# Autodesk Inventor assembly: onlyrobot
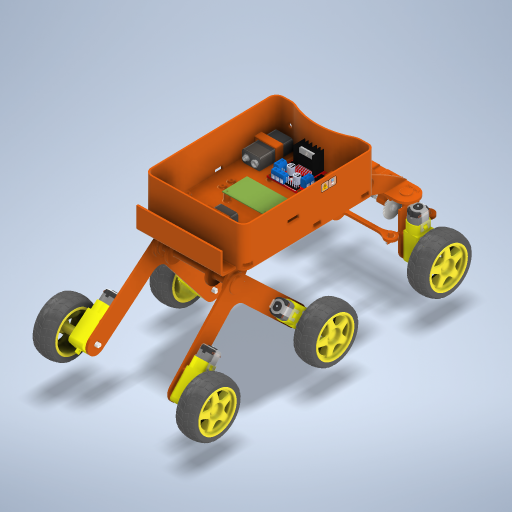
[picture p0: Inventor's stored thumbnail of the model, 512x512]
Saved by Autodesk Inventor 2023.2 (Build 272271000, 271)
## iProperties
Created: 2022-12-08
Part Number: onlyrobot
Document SubType Name: Assembly
Designer: omrfrkmll
Author: omrfrkmll
## Documents named in this file (33)
- C:\Users\omr_f\Desktop\mechanism design project\onlyrobot.iam
- C:\Users\omr_f\Desktop\mechanism design project\robotbase.ipt
- C:\Users\omr_f\Desktop\mechanism design project\sol arka bacak.ipt
- C:\Users\omr_f\Desktop\mechanism design project\6v dc torque motor.iam
- C:\Users\omr_f\Desktop\mechanism design project\Wheel D65x25.ipt
- C:\Users\omr_f\Desktop\mechanism design project\ön sol bacak.ipt
- C:\Users\omr_f\Desktop\mechanism design project\ön sol bacak_MIR.ipt
- C:\Users\omr_f\Desktop\mechanism design project\bişeyleramabendeisimveremedim.ipt
- C:\Users\omr_f\Desktop\mechanism design project\pin.ipt
- C:\Users\omr_f\Desktop\mechanism design project\pintutucu.ipt
- C:\Users\omr_f\Desktop\mechanism design project\pintutucu_MIR.ipt
- C:\Users\omr_f\Desktop\mechanism design project\bilmemç.ipt
- C:\Users\omr_f\Desktop\mechanism design project\Moteur - Moteur.ipt
- C:\Users\omr_f\Desktop\mechanism design project\screw.ipt
- C:\Users\omr_f\Desktop\mechanism design project\dişli.ipt
- C:\Users\omr_f\Desktop\mechanism design project\somun.ipt
- C:\Users\omr_f\Desktop\mechanism design project\benniyebuçüklerinsiminibilmiyorum.ipt
- C:\Users\omr_f\Desktop\mechanism design project\ufakpin.ipt
- C:\Users\omr_f\Desktop\mechanism design project\rockerbogieçükü.ipt
- C:\Users\omr_f\Desktop\mechanism design project\6v dc torque motor_MIR.iam
- C:\Users\omr_f\Desktop\mechanism design project\Wheel D65x25_MIR.ipt
- C:\Users\omr_f\Desktop\mechanism design project\rockerbogieçükü_MIR.ipt
- C:\Users\omr_f\Desktop\mechanism design project\çıkçık.ipt
- C:\Users\omr_f\Desktop\mechanism design project\çıkçıkkarşılıkk.ipt
- C:\Users\omr_f\Desktop\mechanism design project\L298N Driver DC Motor.ipt
- C:\Users\omr_f\Desktop\mechanism design project\devre kartı.ipt
- C:\Users\omr_f\Desktop\mechanism design project\9 Volt Battery.ipt
- C:\Users\omr_f\Desktop\mechanism design project\direksiyon mili tutucu.ipt
- C:\Users\omr_f\Desktop\mechanism design project\şaftuzun.ipt
- C:\Users\omr_f\Desktop\mechanism design project\ön differansiyel.ipt
- C:\Users\omr_f\Desktop\mechanism design project\sol arka bacak_MIR.ipt
- C:\Users\omr_f\Desktop\mechanism design project\onlyrobot\Design Accelerator\Spur Gears2.iam
- C:\Users\omr_f\Desktop\mechanism design project\destek bağlantısı.ipt
## Components (50 placed, 32 different names)
1. robotbase:1 — Mate:87, Mate:88, Mate:89, Mate:90, Mate:91, Mate:92, Mate:94, Mate:95, Mate:96, Mate:97, Mate:99, Mate:100, Mate:101, Mate:102, Mate:103, Mate:113, Mate:114, Mate:115, Mate:120, Mate:121, Mate:122
2. 6v dc torque motor:1 [sub-assembly]
3. Wheel D65x25:1
4. ön sol bacak:1 — Mate:126
5. ön sol bacak_MIR:1 — Mate:133
6. 6v dc torque motor:2 [sub-assembly]
7. Wheel D65x25:2
8. bişeyleramabendeisimveremedim:1 — Flush:1
9. pin:1
10. pintutucu:1 — Mate:106, Mate:110, Mate:111, Mate:112
11. pintutucu_MIR:1 — Mate:105, Mate:109
12. pin:2
13. bilmemç:1 — Mate:104, Mate:105, Mate:106, Mate:112
14. 6v dc torque motor:3 [sub-assembly]
15. Wheel D65x25:3
16. Moteur - Moteur:1 — Flush:1, Mate:130, Flush:3
17. screw:1 — Mate:98, Flush:2, Mate:128, Mate:129
18. dişli:1
19. somun:1
20. benniyebuçüklerinsiminibilmiyorum:1
21. ufakpin:1 — Mate:104
22. rockerbogieçükü:1 — Mate:123
23. 6v dc torque motor:4 [sub-assembly]
24. Wheel D65x25:4
25. 6v dc torque motor_MIR:1 [sub-assembly]
26. Wheel D65x25_MIR:1
27. rockerbogieçükü_MIR:1 — Mate:118
28. 6v dc torque motor_MIR:2 [sub-assembly]
29. Wheel D65x25_MIR:2
30. çıkçık:1 — Mate:117, Mate:124
31. çıkçıkkarşılıkk:1 — Mate:107
32. L298N Driver DC Motor:1 — Mate:90, Mate:91
33. L298N Driver DC Motor:2 — Mate:87, Mate:88
34. L298N Driver DC Motor:3 — Mate:89, Mate:92
35. çıkçık:2
36. çıkçıkkarşılıkk:2 — Mate:116, Mate:119
37. devre kartı:1 — Mate:94, Mate:95, Mate:96
38. 9 Volt Battery:1 — Mate:97, Mate:101
39. direksiyon mili tutucu:1 — Mate:98, Flush:2
40. 9 Volt Battery:2 — Mate:99, Mate:102
41. 9 Volt Battery:3 — Mate:100, Mate:103
42. şaftuzun:1 — Mate:107, Mate:116, Mate:117, Mate:124, Mate:131
43. ön differansiyel:1 — Mate:109, Mate:110, Mate:111
44. sol arka bacak:1 — Mate:113, Mate:114, Mate:115, Mate:118, Mate:119
45. sol arka bacak_MIR:1 — Mate:120, Mate:121, Mate:122, Mate:123
46. çıkçık:3 — Mate:127
47. çıkçıkkarşılıkk:3 — Mate:126, Mate:127
48. Spur Gears:1 [sub-assembly] — Mate:128, Mate:129, Mate:130, Flush:3
49. destek bağlantısı:1 — Mate:131
50. destek bağlantısı:2 — Mate:133
## Relationships (115: Mate 112, Flush 3)
- [Mate]: 6v dc torque motor:1 ↔ Wheel D65x25:1
- [Mate]: 6v dc torque motor:1 ↔ Wheel D65x25:1
- [Mate]: robotbase:1 ↔ ön sol bacak:1
- [Mate]: robotbase:1 ↔ ön sol bacak:1
- [Mate]: robotbase:1 ↔ ön sol bacak:1
- [Mate]: robotbase:1 ↔ ön sol bacak_MIR:1
- [Mate]: robotbase:1 ↔ ön sol bacak_MIR:1
- [Mate]: robotbase:1 ↔ ön sol bacak_MIR:1
- [Mate]: 6v dc torque motor:2 ↔ Wheel D65x25:2
- [Mate]: 6v dc torque motor:2 ↔ Wheel D65x25:2
- [Mate]: ön sol bacak_MIR:1 ↔ bişeyleramabendeisimveremedim:1
- [Mate]: ön sol bacak_MIR:1 ↔ bişeyleramabendeisimveremedim:1
- [Mate]: ön sol bacak_MIR:1 ↔ bişeyleramabendeisimveremedim:1
- [Mate]: bişeyleramabendeisimveremedim:1 ↔ pin:1
- [Mate]: bişeyleramabendeisimveremedim:1 ↔ pin:1
- [Mate]: pin:1 ↔ pintutucu:1
- [Mate]: pin:1 ↔ pintutucu:1
- [Mate]: 6v dc torque motor:2 ↔ pintutucu:1
- [Mate]: pin:1 ↔ pintutucu:1
- [Mate]: 6v dc torque motor:2 ↔ pintutucu:1
- [Mate]: 6v dc torque motor:2 ↔ pintutucu:1
- [Mate]: bişeyleramabendeisimveremedim:1 ↔ pin:2
- [Mate]: bişeyleramabendeisimveremedim:1 ↔ pin:2
- [Mate]: pintutucu_MIR:1 ↔ pin:2
- [Mate]: pintutucu_MIR:1 ↔ pin:2
- [Mate]: pintutucu_MIR:1 ↔ pin:2
- [Mate]: 6v dc torque motor:3 ↔ Wheel D65x25:3
- [Mate]: 6v dc torque motor:3 ↔ Wheel D65x25:3
- [Mate]: pintutucu_MIR:1 ↔ 6v dc torque motor:3
- [Mate]: pintutucu_MIR:1 ↔ 6v dc torque motor:3
- [Mate]: pintutucu_MIR:1 ↔ 6v dc torque motor:3
- [Mate]: bişeyleramabendeisimveremedim:1 ↔ Moteur - Moteur:1
- [Mate]: bişeyleramabendeisimveremedim:1 ↔ Moteur - Moteur:1
- [Mate]: screw:1 ↔ dişli:1
- [Mate]: screw:1 ↔ dişli:1
- [Mate] (7 mm): Moteur - Moteur:1 ↔ dişli:1
- [Mate]: bişeyleramabendeisimveremedim:1 ↔ screw:1
- [Mate]: screw:1 ↔ somun:1
- [Mate]: somun:1 ↔ benniyebuçüklerinsiminibilmiyorum:1
- [Mate]: somun:1 ↔ benniyebuçüklerinsiminibilmiyorum:1
- [Mate]: 6v dc torque motor:2 ↔ pintutucu:1
- [Mate]: 6v dc torque motor:2 ↔ pintutucu:1
- [Mate]: 6v dc torque motor:1 ↔ rockerbogieçükü:1
- [Mate]: 6v dc torque motor:1 ↔ rockerbogieçükü:1
- [Mate]: 6v dc torque motor:1 ↔ rockerbogieçükü:1
- [Mate]: 6v dc torque motor:4 ↔ Wheel D65x25:4
- [Mate]: 6v dc torque motor:4 ↔ Wheel D65x25:4
- [Mate]: rockerbogieçükü:1 ↔ 6v dc torque motor:4
- [Mate]: rockerbogieçükü:1 ↔ 6v dc torque motor:4
- [Mate]: rockerbogieçükü:1 ↔ 6v dc torque motor:4
- [Mate]: 6v dc torque motor_MIR:1 ↔ Wheel D65x25_MIR:1
- [Mate]: 6v dc torque motor_MIR:1 ↔ Wheel D65x25_MIR:1
- [Mate]: 6v dc torque motor_MIR:1 ↔ rockerbogieçükü_MIR:1
- [Mate]: 6v dc torque motor_MIR:1 ↔ rockerbogieçükü_MIR:1
- [Mate]: 6v dc torque motor_MIR:1 ↔ rockerbogieçükü_MIR:1
- [Mate]: rockerbogieçükü_MIR:1 ↔ 6v dc torque motor_MIR:2
- [Mate]: rockerbogieçükü_MIR:1 ↔ 6v dc torque motor_MIR:2
- [Mate]: rockerbogieçükü_MIR:1 ↔ 6v dc torque motor_MIR:2
- [Mate]: 6v dc torque motor_MIR:2 ↔ Wheel D65x25_MIR:2
- [Mate]: 6v dc torque motor_MIR:2 ↔ Wheel D65x25_MIR:2
- [Mate]: rockerbogieçükü:1 ↔ çıkçık:1
- [Mate]: rockerbogieçükü:1 ↔ çıkçık:1
- [Mate]: çıkçık:1 ↔ çıkçıkkarşılıkk:1
- [Mate]: bilmemç:1 ↔ ufakpin:1
- [Mate]: rockerbogieçükü_MIR:1 ↔ çıkçık:2
- [Mate]: rockerbogieçükü_MIR:1 ↔ çıkçıkkarşılıkk:2
- [Mate]: rockerbogieçükü_MIR:1 ↔ çıkçık:2
- [Mate]: çıkçık:2 ↔ çıkçıkkarşılıkk:2
- Mate:87: robotbase:1 ↔ L298N Driver DC Motor:2
- Mate:88: robotbase:1 ↔ L298N Driver DC Motor:2
- Mate:89: robotbase:1 ↔ L298N Driver DC Motor:3
- Mate:90: robotbase:1 ↔ L298N Driver DC Motor:1
- Mate:91: robotbase:1 ↔ L298N Driver DC Motor:1
- Mate:92: robotbase:1 ↔ L298N Driver DC Motor:3
- Flush:1: bişeyleramabendeisimveremedim:1 ↔ Moteur - Moteur:1
- Mate:94: robotbase:1 ↔ devre kartı:1
- Mate:95: robotbase:1 ↔ devre kartı:1
- Mate:96: robotbase:1 ↔ devre kartı:1
- Mate:97: robotbase:1 ↔ 9 Volt Battery:1
- Mate:98: screw:1 ↔ direksiyon mili tutucu:1
- Flush:2: screw:1 ↔ direksiyon mili tutucu:1
- Mate:99: robotbase:1 ↔ 9 Volt Battery:2
- Mate:100: robotbase:1 ↔ 9 Volt Battery:3
- Mate:101: robotbase:1 ↔ 9 Volt Battery:1
- Mate:102: robotbase:1 ↔ 9 Volt Battery:2
- Mate:103: robotbase:1 ↔ 9 Volt Battery:3
- Mate:104: bilmemç:1 ↔ ufakpin:1
- Mate:105: pintutucu_MIR:1 ↔ bilmemç:1
- Mate:106: pintutucu:1 ↔ bilmemç:1
- Mate:107: çıkçıkkarşılıkk:1 ↔ şaftuzun:1
- Mate:109: pintutucu_MIR:1 ↔ ön differansiyel:1
- Mate:110: pintutucu:1 ↔ ön differansiyel:1
- Mate:111: pintutucu:1 ↔ ön differansiyel:1
- Mate:112: pintutucu:1 ↔ bilmemç:1
- Mate:113: robotbase:1 ↔ sol arka bacak:1
- Mate:114: robotbase:1 ↔ sol arka bacak:1
- Mate:115: robotbase:1 ↔ sol arka bacak:1
- Mate:116: çıkçıkkarşılıkk:2 ↔ şaftuzun:1
- Mate:117: çıkçık:1 ↔ şaftuzun:1
- Mate:118: rockerbogieçükü_MIR:1 ↔ sol arka bacak:1
- Mate:119: çıkçıkkarşılıkk:2 ↔ sol arka bacak:1
- Mate:120: robotbase:1 ↔ sol arka bacak_MIR:1
- Mate:121: robotbase:1 ↔ sol arka bacak_MIR:1
- Mate:122: robotbase:1 ↔ sol arka bacak_MIR:1
- Mate:123: rockerbogieçükü:1 ↔ sol arka bacak_MIR:1
- Mate:124 (2 mm): çıkçık:1 ↔ şaftuzun:1
- [Mate]: çıkçık:3 ↔ çıkçıkkarşılıkk:3
- Mate:126: ön sol bacak:1 ↔ çıkçıkkarşılıkk:3
- Mate:127: çıkçık:3 ↔ çıkçıkkarşılıkk:3
- Mate:128: screw:1 ↔ Spur Gears:1
- Mate:129: screw:1 ↔ Spur Gears:1
- Mate:130: Moteur - Moteur:1 ↔ Spur Gears:1
- Flush:3: Moteur - Moteur:1 ↔ Spur Gears:1
- Mate:131: şaftuzun:1 ↔ destek bağlantısı:1
- Mate:133: ön sol bacak_MIR:1 ↔ destek bağlantısı:2
## Named parameters: d156_d59_d45 = 0 mm, d157_d60_d46 = 0 mm, d100_d59_d45 = 0 mm, d101_d60_d46 = 0 mm, d59_d45 = 0 mm, d60_d46 = 0 mm, d59_d65 = 0 mm, d60_d68 = 0 mm, d61_d69 = 0 mm, d62_d70 = 0 mm, d63_d71 = 0 mm, d64_d72 = 0 mm, d77_d45 = 0 mm, d78_d46 = 0 mm, d67_d79 = 0 mm, d68_d80 = 0 mm, d69_d81 = 0 mm, d70_d82 = 0 mm, d71_d83 = 0 mm, d72_d85 = 0 mm, d172_d196 = 0 mm
